# Autodesk Inventor assembly: Camera system
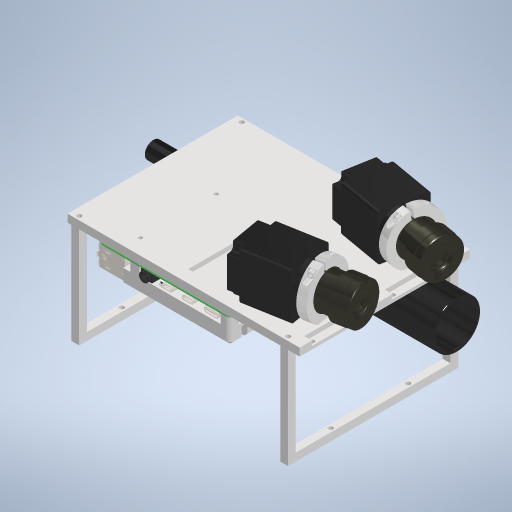
[picture p0: Inventor's stored thumbnail of the model, 512x512]
Saved by Autodesk Inventor 2023 (Build 270158000, 158)
## iProperties
Created: 2023-04-08
Part Number: Camera system
Document SubType Name: Assembly
Designer: ASARe-DAQ-PC
Author: ASARe-DAQ-PC
## Documents named in this file (7)
- D:\EB camera\model of EB camera\for manufacture\Camera system.iam
- D:\EB camera\model of EB camera\for manufacture\Camera plate.ipt
- D:\EB camera\model of EB camera\for manufacture\EVK4 – HD.iam
- D:\EB camera\model of EB camera\for manufacture\Camera plate shell.ipt
- D:\EB camera\model of EB camera\for manufacture\Raspberry Pi 4B with heatsink.iam
- D:\EB camera\model of EB camera\for manufacture\Power bank.iam
- D:\EB camera\model of EB camera\for manufacture\Laser.iam
## Components (8 placed, 6 different names)
1. Camera plate:1 — Angle:1, Mate:7, Insert:13, Insert:14, Insert:15, Insert:16, Mate:10, Insert:18, Insert:19, Insert:20, Insert:21, Mate:11
2. EVK4 – HD:1 [sub-assembly] — Angle:1, Mate:7, Angle:2
3. Camera plate shell:1 — Insert:13, Insert:14
4. Camera plate shell:2 — Insert:15, Insert:16
5. Raspberry Pi 4B with heatsink:1 [sub-assembly] — Mate:10, Insert:18, Insert:19, Insert:20, Insert:21
6. Power bank:1 [sub-assembly]
7. Laser:1 [sub-assembly]
8. EVK4 – HD:2 [sub-assembly] — Mate:11, Angle:2
## Relationships (13: Insert 8, Mate 3, Angle 2)
- Angle:1 (180 deg): Camera plate:1 ↔ EVK4 – HD:1
- Mate:7: Camera plate:1 ↔ EVK4 – HD:1
- Insert:13: Camera plate:1 ↔ Camera plate shell:1
- Insert:14: Camera plate:1 ↔ Camera plate shell:1
- Insert:15: Camera plate:1 ↔ Camera plate shell:2
- Insert:16: Camera plate:1 ↔ Camera plate shell:2
- Mate:10: Camera plate:1 ↔ Raspberry Pi 4B with heatsink:1
- Insert:18 (2 mm): Camera plate:1 ↔ Raspberry Pi 4B with heatsink:1
- Insert:19 (2 mm): Camera plate:1 ↔ Raspberry Pi 4B with heatsink:1
- Insert:20 (2 mm): Camera plate:1 ↔ Raspberry Pi 4B with heatsink:1
- Insert:21 (2 mm): Camera plate:1 ↔ Raspberry Pi 4B with heatsink:1
- Mate:11: Camera plate:1 ↔ EVK4 – HD:2
- Angle:2 (160 deg): EVK4 – HD:1 ↔ EVK4 – HD:2
